# Autodesk Inventor assembly: magazine
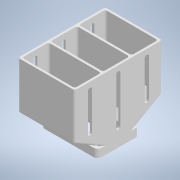
[picture p0: Inventor's stored thumbnail of the model, 180x180]
Saved by Autodesk Inventor 2021 (Build 250183000, 183)
## iProperties
Created: 2024-03-18
Part Number: magazine
Document SubType Name: Assembly
Designer: 22hamfri
Author: 22hamfri
## Documents named in this file (3)
- C:\Users\22hamfri\Documents\School\Programmering\domino-bil\CAD\magazine.iam
- C:\Users\22hamfri\Documents\School\Programmering\domino-bil\CAD\magazine-adapter.ipt
- C:\Users\22hamfri\Documents\School\Programmering\domino-bil\CAD\magazine-tower.ipt
## Components (2 placed, 2 different names)
1. magazine-adapter:1 — Rigid:1
2. magazine-tower:1 — Rigid:1
## Relationships (1: WeldJoint 1)
- Rigid:1 [WeldJoint]: magazine-adapter:1 ↔ magazine-tower:1
